# Autodesk Inventor assembly: module
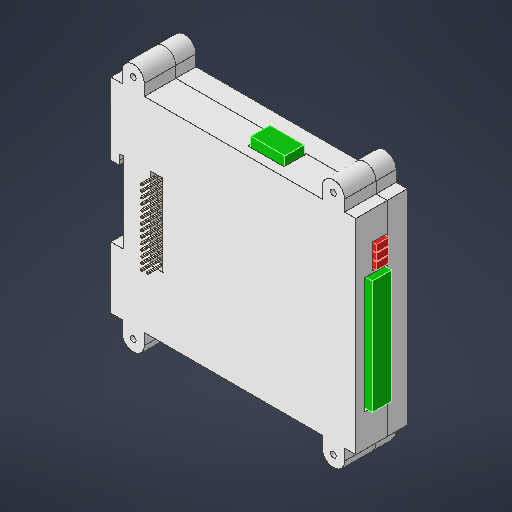
[picture p0: Inventor's stored thumbnail of the model, 512x512]
Saved by Autodesk Inventor 2025 (Build 290162000, 162)
## iProperties
Created: 2024-08-31
Part Number: module
Document SubType Name: Assembly
Designer: Dawid
Author: Dawid
## Documents named in this file (4)
- C:\Users\Dawid\Desktop\Magisterka\plc_io_module_case\module.iam
- C:\Users\Dawid\Desktop\Magisterka\plc_io_module_case\plc_io_module.ipt
- C:\Users\Dawid\Desktop\Magisterka\plc_io_module_case\module_case.ipt
- module_case.ipt
## Components (2 placed, 2 different names)
1. plc_io_module.ipt:1 — Rigid:1
2. module_base.ipt:1 — Rigid:1
## Relationships (1: WeldJoint 1)
- Rigid:1 [WeldJoint]: plc_io_module.ipt:1 ↔ module_base.ipt:1
